# Autodesk Inventor assembly: CollectorHolderAssembly
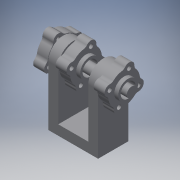
[picture p0: Inventor's stored thumbnail of the model, 180x180]
Saved by Autodesk Inventor 2017 (Build 210142000, 142)
## iProperties
Created: 2017-04-19
Part Number: CollectorHolderAssembly
Document SubType Name: Assembly
Designer: User
Author: User
## Documents named in this file (5)
- C:\Robotics\CAD\2016-17_CAD\CollectorHolderAssembly.iam
- C:\Robotics\CAD\2016-17_CAD\CollectorHolder.ipt
- C:\Robotics\CAD\2016-17_CAD\Axle2.11.ipt
- C:\Robotics\CAD\COTSParts\Actobotics\535 parts\535198.ipt
- C:\Robotics\CAD\COTSParts\Actobotics\545 parts\545556.ipt
## Components (7 placed, 4 different names)
1. CollectorHolder:1 — Insert:1, Insert:2, Insert:3, Insert:4, Insert:5
2. Axle2.11:1 — Insert:3
3. 535198:1 — Insert:1, Insert:6
4. 535198:2 — Insert:2
5. 545556:1 — Insert:4
6. 545556:2 — Insert:5
7. 545556:3 — Insert:6
## Relationships (6: Insert 6)
- Insert:1: CollectorHolder:1 ↔ 535198:1
- Insert:2: CollectorHolder:1 ↔ 535198:2
- Insert:3 (-9.779 mm): CollectorHolder:1 ↔ Axle2.11:1
- Insert:4: CollectorHolder:1 ↔ 545556:1
- Insert:5: CollectorHolder:1 ↔ 545556:2
- Insert:6: 535198:1 ↔ 545556:3
